# Autodesk Inventor assembly: Vacio
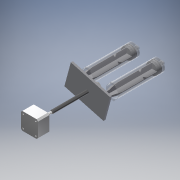
[picture p0: Inventor's stored thumbnail of the model, 180x180]
Saved by Autodesk Inventor 2018.3 (Build 223284000, 284)
## iProperties
Created: 2019-02-28
Part Number: Vacio
Document SubType Name: Assembly
Designer: Mario
Author: Mario
## Documents named in this file (7)
- C:\Users\Mario\Documents\Inventor\Underwater glider\Vacio.iam
- C:\Users\Mario\Documents\Inventor\Underwater glider\Motor.ipt
- C:\Users\Mario\Documents\Inventor\Underwater glider\Jeringa core.ipt
- C:\Users\Mario\Documents\Inventor\Underwater glider\Jeringa shell.ipt
- C:\Users\Mario\Documents\Inventor\Underwater glider\Valvula.ipt
- C:\Users\Mario\Documents\Inventor\Underwater glider\jalador.ipt
- C:\Users\Mario\Documents\Inventor\Content Center Files\R2018\en-US\DIN 933\DIN 933 - M8  x 110.ipt
## Components (9 placed, 6 different names)
1. Motor:1 — Cylindrical:5
2. Jeringa core:1 — Mate:2, Cylindrical:2, Mate:3
3. Jeringa shell:1 — Cylindrical:3, Flush:1
4. Jeringa core:2 — Mate:1, Cylindrical:1, Mate:4
5. Jeringa shell:2 — Cylindrical:4, Flush:1
6. Valvula:1 — Mate:1, Cylindrical:1, Cylindrical:4
7. Valvula:2 — Mate:2, Cylindrical:2, Cylindrical:3
8. jalador:1 — Mate:3, Mate:4, Cylindrical:6
9. DIN 933 - replaced by DIN EN 24017 M8  x 110:1 — Cylindrical:5, Cylindrical:6
## Relationships (11: CylindricalJoint 6, Mate 4, Flush 1)
- Mate:1: Jeringa core:2 ↔ Valvula:1
- Mate:2: Jeringa core:1 ↔ Valvula:2
- Cylindrical:1: Jeringa core:2 ↔ Valvula:1
- Cylindrical:2: Jeringa core:1 ↔ Valvula:2
- Cylindrical:3: Jeringa shell:1 ↔ Valvula:2
- Cylindrical:4: Jeringa shell:2 ↔ Valvula:1
- Mate:3: Jeringa core:1 ↔ jalador:1
- Mate:4: Jeringa core:2 ↔ jalador:1
- Cylindrical:5: Motor:1 ↔ DIN 933 - replaced by DIN EN 24017 M8  x 110:1
- Cylindrical:6: jalador:1 ↔ DIN 933 - replaced by DIN EN 24017 M8  x 110:1
- Flush:1: Jeringa shell:1 ↔ Jeringa shell:2
